# Autodesk Inventor assembly: Multilegged
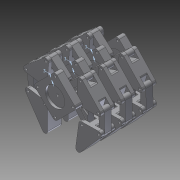
[picture p0: Inventor's stored thumbnail of the model, 180x180]
Saved by Autodesk Inventor 2011 SP2 (Build 150309200, 309)
## iProperties
Created: 2014-05-26
Part Number: Multilegged
Document SubType Name: Assembly
Designer: Maurice Woods
Author: Maurice Woods
## Documents named in this file (3)
- C:\Users\Maurice\Documents\GitHub\strandbeest\Multilegged.iam
- C:\Users\Maurice\Documents\GitHub\strandbeest\MasterAssembly.iam
- C:\Users\Maurice\Documents\GitHub\strandbeest\MatingPlates.ipt
## Components (4 placed, 2 different names)
1. MasterAssembly:1 [sub-assembly] — Mate:1, Mate:2, Mate:4
2. MasterAssembly:2 [sub-assembly] — Mate:1, Mate:2, Mate:3, Mate:4, Mate:5, Mate:6
3. MasterAssembly:3 [sub-assembly] — Mate:3, Mate:5, Mate:6, Mate:7, Mate:8, Mate:9
4. MatingPlates:1 — Mate:7, Mate:8, Mate:9
## Relationships (9: Mate 9)
- Mate:1: MasterAssembly:1 ↔ MasterAssembly:2
- Mate:2 (20 mm): MasterAssembly:1 ↔ MasterAssembly:2
- Mate:3: MasterAssembly:2 ↔ MasterAssembly:3
- Mate:4: MasterAssembly:1 ↔ MasterAssembly:2
- Mate:5: MasterAssembly:2 ↔ MasterAssembly:3
- Mate:6 (20 mm): MasterAssembly:2 ↔ MasterAssembly:3
- Mate:7: MasterAssembly:3 ↔ MatingPlates:1
- Mate:8: MasterAssembly:3 ↔ MatingPlates:1
- Mate:9: MasterAssembly:3 ↔ MatingPlates:1
